# Autodesk Inventor assembly: PCB_Case
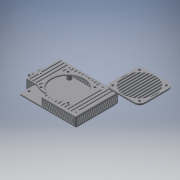
[picture p0: Inventor's stored thumbnail of the model, 180x180]
Saved by Autodesk Inventor 2019.3 (Build 233278000, 278)
## iProperties
Created: 2020-10-08
Part Number: PCB_Case
Material: Generisch
Document SubType Name: Assembly
Designer: Nicolas Frick
Author: Nicolas Frick
## Documents named in this file (5)
- C:\Users\Nicolas Frick\Sync\OneDrive\airhockeybot\mechanical_design\inventor\PCB_Case.iam
- C:\Users\Nicolas Frick\Sync\OneDrive\airhockeybot\mechanical_design\inventor\PCB_Cover.ipt
- C:\Users\Nicolas Frick\Sync\OneDrive\airhockeybot\mechanical_design\inventor\PCB_Case_Btm.ipt
- C:\Users\Nicolas Frick\Sync\OneDrive\airhockeybot\mechanical_design\inventor\Fan_blend.ipt
- C:\Users\Nicolas Frick\Sync\OneDrive\airhockeybot\mechanical_design\inventor\Reset_beam.ipt
## Components (4 placed, 4 different names)
1. PCB_Cover:1 — Passend:5, Passend:6, Passend:7, Fluchtend:3, Passend:8, Passend:9
2. PCB_Case_Btm:1 — Passend:3, Passend:4, Fluchtend:2, Passend:5, Passend:6, Passend:7
3. Fan_blend:1 — Fluchtend:3
4. Reset_beam:1 — Passend:8, Passend:9
## Relationships (9: Mate 7, Flush 2)
- Passend:3 [Mate]: PCB_Case_Btm:1
- Passend:4 [Mate]: PCB_Case_Btm:1
- Fluchtend:2 [Flush]: PCB_Case_Btm:1
- Passend:5 [Mate]: PCB_Cover:1 ↔ PCB_Case_Btm:1
- Passend:6 [Mate]: PCB_Cover:1 ↔ PCB_Case_Btm:1
- Passend:7 [Mate]: PCB_Cover:1 ↔ PCB_Case_Btm:1
- Fluchtend:3 [Flush]: PCB_Cover:1 ↔ Fan_blend:1
- Passend:8 [Mate]: PCB_Cover:1 ↔ Reset_beam:1
- Passend:9 [Mate]: PCB_Cover:1 ↔ Reset_beam:1
